# Autodesk Inventor assembly: SLIDE,TOP,ELEVATOR,STAGE1,LH
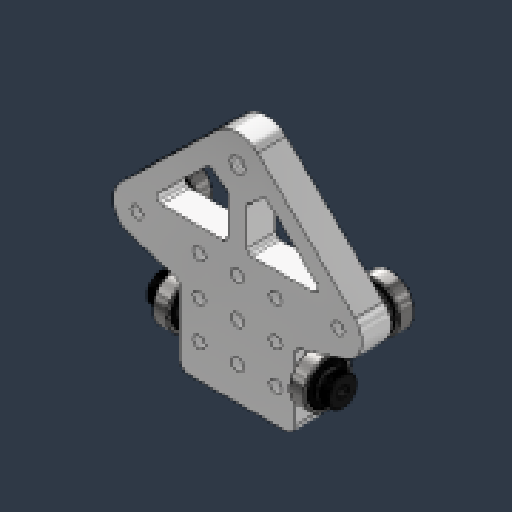
[picture p0: Inventor's stored thumbnail of the model, 512x512]
Saved by Autodesk Inventor 2024.3 (Build 283343000, 343)
## iProperties
Category: _
Manager: _
ILogicPurgeVersion: 3.4.1.0
ILogicPurgeAssembly: InventorDocumentWrapper
OnSaveVersion: 3.4.3.0
OnSaveAssembly: COREAutomationManager
Created: 2025-01-27
Part Number: SLIDE,TOP,ELEVATOR,STAGE1,LH
Checked By: 00
Engr Approved By: _
User Status: Work In Process
Description: ASSY,STANDARD (mm)
Document SubType Name: Assembly
Mfg Approved By: John.Thibert
Designer: John.Thibert
CN_MASS: 0.0
CN_SERVICEABLE: _
FIRST_DESCRIPTION: _
SECOND_DESCRIPTION: _
THIRD_DESCRIPTION: _
CL_runCount: 0
ModelCat: Uncategorized
Subject: _
Author: John.Thibert
Keywords: -
Revision Number: A
## Documents named in this file (7)
- C:\Users\Jthib\OneDrive\Robotics\4_Robot Files - 2025 - Poseidon\Elevator\SLIDE,TOP,ELEVATOR,STAGE1,LH.iam
- C:\Users\Jthib\OneDrive\Robotics\4_Robot Files - 2025 - Poseidon\Elevator\60355K336_Ball Bearing\60355K336_Ball Bearing\60355K336_Ball Bearing.ipt
- C:\Users\Jthib\OneDrive\Robotics\4_Robot Files - 2025 - Poseidon\Fasteners\91259A171_Alloy Steel Shoulder Screw\91259A171_Alloy Steel Shoulder Screw\91259A171_Alloy Steel Shoulder Screw.ipt
- C:\Users\Jthib\OneDrive\Robotics\4_Robot Files - 2025 - Poseidon\Elevator\SPACER,BEARING,SLIDE,THIN,ELEVATOR.ipt
- C:\Users\Jthib\OneDrive\Robotics\4_Robot Files - 2025 - Poseidon\Elevator\PLATE,TOP,ELEVATOR,STAGE1.ipt
- C:\Users\Jthib\OneDrive\Robotics\4_Robot Files - 2025 - Poseidon\Fasteners\90318A505_Ultra-Low-Profile Precision Shoulder Screw\90318A505_Ultra-Low-Profile Precision Shoulder Screw\90318A505_Ultra-Low-Pr.ipt
- C:\Users\Jthib\OneDrive\Robotics\4_Robot Files - 2025 - Poseidon\Elevator\SPACER,BEARING,SLIDE,TOP,ELEVATOR.ipt
## Components (15 placed, 6 different names)
1. PLATE,TOP,ELEVATOR,STAGE1.ipt:1 — Mate:13, Mate:15, Flush:1, Insert:8, Insert:11, Insert:13, Insert:14
2. 60355K336_Ball Bearing.ipt:1 — Insert:7
3. 91259A171_Alloy Steel Shoulder Screw.ipt:1 — Insert:8, Mate:24
4. SPACER,BEARING,SLIDE,THIN,ELEVATOR.ipt:1 — Mate:24
5. SPACER,BEARING,SLIDE,THIN,ELEVATOR.ipt:2 — Insert:7
6. 60355K336_Ball Bearing.ipt:2 — Mate:26
7. 91259A171_Alloy Steel Shoulder Screw.ipt:2 — Mate:26, Insert:11
8. SPACER,BEARING,SLIDE,THIN,ELEVATOR.ipt:3
9. SPACER,BEARING,SLIDE,THIN,ELEVATOR.ipt:4
10. 60355K336_Ball Bearing.ipt:3
11. SPACER,BEARING,SLIDE,TOP,ELEVATOR.ipt:1
12. 90318A505_Ultra-Low-Pr.ipt:1 — Insert:13
13. 60355K336_Ball Bearing.ipt:4
14. SPACER,BEARING,SLIDE,TOP,ELEVATOR.ipt:2
15. 90318A505_Ultra-Low-Pr.ipt:2 — Insert:14
## Relationships (23: Mate 14, Insert 8, Flush 1)
- Mate:13: PLATE,TOP,ELEVATOR,STAGE1.ipt:1
- Mate:15: PLATE,TOP,ELEVATOR,STAGE1.ipt:1
- Flush:1: PLATE,TOP,ELEVATOR,STAGE1.ipt:1
- [Mate]: PLATE,TOP,ELEVATOR,STAGE1.ipt:1 ↔ 60355K336_Ball Bearing.ipt:1
- [Insert]: 60355K336_Ball Bearing.ipt:1 ↔ SPACER,BEARING,SLIDE,THIN,ELEVATOR.ipt:1
- Insert:7: 60355K336_Ball Bearing.ipt:1 ↔ SPACER,BEARING,SLIDE,THIN,ELEVATOR.ipt:2
- Insert:8: PLATE,TOP,ELEVATOR,STAGE1.ipt:1 ↔ 91259A171_Alloy Steel Shoulder Screw.ipt:1
- Mate:24: 91259A171_Alloy Steel Shoulder Screw.ipt:1 ↔ SPACER,BEARING,SLIDE,THIN,ELEVATOR.ipt:1
- [Insert]: 60355K336_Ball Bearing.ipt:2 ↔ SPACER,BEARING,SLIDE,THIN,ELEVATOR.ipt:3
- [Insert]: 60355K336_Ball Bearing.ipt:2 ↔ SPACER,BEARING,SLIDE,THIN,ELEVATOR.ipt:4
- [Mate]: 91259A171_Alloy Steel Shoulder Screw.ipt:2 ↔ SPACER,BEARING,SLIDE,THIN,ELEVATOR.ipt:3
- Mate:26: 60355K336_Ball Bearing.ipt:2 ↔ 91259A171_Alloy Steel Shoulder Screw.ipt:2
- Insert:11: PLATE,TOP,ELEVATOR,STAGE1.ipt:1 ↔ 91259A171_Alloy Steel Shoulder Screw.ipt:2
- [Mate]: 60355K336_Ball Bearing.ipt:3 ↔ 90318A505_Ultra-Low-Pr.ipt:1
- [Mate]: 60355K336_Ball Bearing.ipt:3 ↔ 90318A505_Ultra-Low-Pr.ipt:1
- [Mate]: SPACER,BEARING,SLIDE,TOP,ELEVATOR.ipt:1 ↔ 90318A505_Ultra-Low-Pr.ipt:1
- [Mate]: 60355K336_Ball Bearing.ipt:3 ↔ SPACER,BEARING,SLIDE,TOP,ELEVATOR.ipt:1
- Insert:13: PLATE,TOP,ELEVATOR,STAGE1.ipt:1 ↔ 90318A505_Ultra-Low-Pr.ipt:1
- [Mate]: 60355K336_Ball Bearing.ipt:4 ↔ 90318A505_Ultra-Low-Pr.ipt:2
- [Mate]: 60355K336_Ball Bearing.ipt:4 ↔ 90318A505_Ultra-Low-Pr.ipt:2
- [Mate]: SPACER,BEARING,SLIDE,TOP,ELEVATOR.ipt:2 ↔ 90318A505_Ultra-Low-Pr.ipt:2
- [Mate]: 60355K336_Ball Bearing.ipt:4 ↔ SPACER,BEARING,SLIDE,TOP,ELEVATOR.ipt:2
- Insert:14: PLATE,TOP,ELEVATOR,STAGE1.ipt:1 ↔ 90318A505_Ultra-Low-Pr.ipt:2
## Named parameters: d49_d352 = 0 mm, d50_d46 = 0 mm, d51_d48 = 0 mm, d75_d70_d65 = 0 mm, d76_d71_d66 = 0 mm, d77_d72_d68 = 0 mm, d78_d73_d69 = 0 mm, d81_d75_d70_d65 = 0 mm, d82_d76_d71_d66 = 0 mm, d83_d77_d72_d68 = 0 mm, d84_d78_d73_d69 = 0 mm
